# Autodesk Inventor assembly: Tractor_Assembly
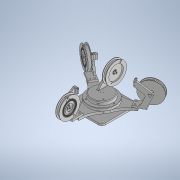
[picture p0: Inventor's stored thumbnail of the model, 180x180]
Saved by Autodesk Inventor 2022 (Build 260153070, 153G)
## iProperties
Created: 2022-03-05
Part Number: Tractor_Assembly
Document SubType Name: Assembly
Designer: a laptop
Author: a laptop
## Documents named in this file (5)
- C:\Users\a laptop\Desktop\MDL_2021_Project\Tractor_Assembly.iam
- C:\Users\a laptop\Desktop\MDL_2021_Project\Tractor_Plates\Tractor_Plates.iam
- C:\Users\a laptop\Desktop\MDL_2021_Project\Return_Spool_Reel\Return_Spool_Mount.iam
- C:\Users\a laptop\Desktop\MDL_2021_Project\AS5600.ipt
- C:\Users\a laptop\Desktop\MDL_2021_Project\Arm_Spool\Arm_Frame.iam
## Components (6 placed, 4 different names)
1. Tractor_Plates:1 [sub-assembly] — Mate:1, Mate:2, Mate:4, Mate:5, Mate:8, Mate:9, Mate:10, Mate:11, Mate:12, Mate:13, Mate:14, Mate:15, Mate:16
2. Return_Spool_Mount:1 [sub-assembly] — Mate:1, Mate:2, Mate:6, Mate:7
3. AS5600:1 — Mate:4, Mate:5, Mate:6, Mate:7
4. Arm_Frame [sub-assembly] — Mate:8, Mate:9, Mate:10
5. Arm_Frame:2 [sub-assembly] — Mate:14, Mate:15, Mate:16
6. Arm_Frame:3 [sub-assembly] — Mate:11, Mate:12, Mate:13
## Relationships (15: Mate 15)
- Mate:1: Tractor_Plates:1 ↔ Return_Spool_Mount:1
- Mate:2: Tractor_Plates:1 ↔ Return_Spool_Mount:1
- Mate:4 (5 mm): Tractor_Plates:1 ↔ AS5600:1
- Mate:5: Tractor_Plates:1 ↔ AS5600:1
- Mate:6: Return_Spool_Mount:1 ↔ AS5600:1
- Mate:7: Return_Spool_Mount:1 ↔ AS5600:1
- Mate:8: Tractor_Plates:1 ↔ Arm_Frame
- Mate:9: Tractor_Plates:1 ↔ Arm_Frame
- Mate:10: Tractor_Plates:1 ↔ Arm_Frame
- Mate:11: Tractor_Plates:1 ↔ Arm_Frame:3
- Mate:12: Tractor_Plates:1 ↔ Arm_Frame:3
- Mate:13: Tractor_Plates:1 ↔ Arm_Frame:3
- Mate:14: Tractor_Plates:1 ↔ Arm_Frame:2
- Mate:15: Tractor_Plates:1 ↔ Arm_Frame:2
- Mate:16: Tractor_Plates:1 ↔ Arm_Frame:2
